# Autodesk Inventor assembly: A000
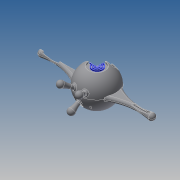
[picture p0: Inventor's stored thumbnail of the model, 180x180]
Saved by Autodesk Inventor 2017 (Build 210142000, 142)
## iProperties
Created: 2018-10-19
Part Number: A000
Document SubType Name: Assembly
Designer: Gilles Mottiez
Description: Prototype v2.0 Visible Energy
Author: Gilles Mottiez
## Documents named in this file (20)
- C:\Users\Gilles Mottiez\Documents\HES\I5_6\PGA\GitHubInventor\visibleEnergy_2.iam
- visibleEnergy_2.iam
- C:\Users\Gilles Mottiez\Documents\HES\I5_6\PGA\GitHubInventor\body_face_modif.ipt
- C:\Users\Gilles Mottiez\Documents\HES\I5_6\PGA\GitHubInventor\plateforme_rpi_servo.iam
- C:\Users\Gilles Mottiez\Documents\HES\I5_6\PGA\GitHubInventor\display_7seg.ipt
- C:\Users\Gilles Mottiez\Documents\HES\I5_6\PGA\GitHubInventor\arbre.ipt
- arbre.ipt
- C:\Users\Gilles Mottiez\Documents\HES\I5_6\PGA\GitHubInventor\palier_face.ipt
- palier_face.ipt
- C:\Users\Gilles Mottiez\Documents\HES\I5_6\PGA\GitHubInventor\body_dos.ipt
- C:\Users\Gilles Mottiez\Documents\HES\I5_6\PGA\GitHubInventor\axe.ipt
- axe.ipt
- C:\Users\Gilles Mottiez\Documents\HES\I5_6\PGA\GitHubInventor\ressort.ipt
- C:\Users\Gilles Mottiez\Documents\HES\I5_6\PGA\GitHubInventor\pieds.ipt
- C:\Users\Gilles Mottiez\Documents\HES\I5_6\PGA\GitHubInventor\bras_osc_dos.ipt
- bras_osc_dos.ipt
- C:\Users\Gilles Mottiez\Documents\HES\I5_6\PGA\GitHubInventor\bras_osc_front.ipt
- C:\Users\Gilles Mottiez\Documents\HES\I5_6\PGA\GitHubInventor\goupille_ressort.ipt
- goupille_ressort.ipt
- C:\Users\Gilles Mottiez\Documents\HES\I5_6\PGA\GitHubInventor\vis_blocage_arbre.ipt
## Components (17 placed, 13 different names)
1. body_face_modif:1 — Placage:1, Placage:2, Logement:1, Logement:2, Logement:4, Placage:3, Logement:9, Logement:11, Placage:6, Logement:22, Angle:3
2. plateforme_rpi_servo:1 [sub-assembly] — Placage:1, Placage:2, Logement:3, Logement:12, Logement:13, Logement:14, Logement:15, Logement:16, Logement:17, Logement:18, Logement:19, Angle:3
3. display_7seg:1 — Logement:1, Logement:2
4. arbre:1 — Logement:3, Logement:8, Placage:4, Placage:5, Logement:21
5. palier_face:1 — Logement:4
6. body_dos:1 — Logement:7, Logement:10, Placage:6, Logement:22, Angle:2
7. axe:1 — Logement:7
8. ressort:1 — Placage:3, Logement:8, Logement:20, Placage:4
9. pieds:1 — Logement:11
10. pieds:2 — Logement:9
11. pieds:3 — Logement:10, Angle:2
12. bras_osc_dos:1 — Logement:16, Logement:17
13. bras_osc_front:2 — Logement:14, Logement:15
14. bras_osc_dos:3 — Logement:18, Logement:19
15. bras_osc_front:4 — Logement:12, Logement:13
16. goupille_ressort:1 — Logement:20
17. vis_blocage_arbre:1 — Placage:5, Logement:21
## Relationships (28: Insert 20, Mate 6, Angle 2)
- Placage:1 [Mate]: body_face_modif:1 ↔ plateforme_rpi_servo:1
- Placage:2 [Mate]: body_face_modif:1 ↔ plateforme_rpi_servo:1
- Logement:1 [Insert]: body_face_modif:1 ↔ display_7seg:1
- Logement:2 [Insert]: body_face_modif:1 ↔ display_7seg:1
- Logement:3 [Insert]: plateforme_rpi_servo:1 ↔ arbre:1
- Logement:4 [Insert]: body_face_modif:1 ↔ palier_face:1
- Logement:7 [Insert]: body_dos:1 ↔ axe:1
- Placage:3 [Mate]: body_face_modif:1 ↔ ressort:1
- Logement:8 [Insert]: arbre:1 ↔ ressort:1
- Logement:9 [Insert]: body_face_modif:1 ↔ pieds:2
- Logement:10 [Insert]: body_dos:1 ↔ pieds:3
- Logement:11 [Insert]: body_face_modif:1 ↔ pieds:1
- Logement:12 [Insert]: plateforme_rpi_servo:1 ↔ bras_osc_front:4
- Logement:13 [Insert]: plateforme_rpi_servo:1 ↔ bras_osc_front:4
- Logement:14 [Insert]: plateforme_rpi_servo:1 ↔ bras_osc_front:2
- Logement:15 [Insert]: plateforme_rpi_servo:1 ↔ bras_osc_front:2
- Logement:16 [Insert]: plateforme_rpi_servo:1 ↔ bras_osc_dos:1
- Logement:17 [Insert]: plateforme_rpi_servo:1 ↔ bras_osc_dos:1
- Logement:18 [Insert]: plateforme_rpi_servo:1 ↔ bras_osc_dos:3
- Logement:19 [Insert]: plateforme_rpi_servo:1 ↔ bras_osc_dos:3
- Logement:20 [Insert]: ressort:1 ↔ goupille_ressort:1
- Placage:4 [Mate]: arbre:1 ↔ ressort:1
- Placage:5 [Mate]: arbre:1 ↔ vis_blocage_arbre:1
- Logement:21 [Insert] (1 mm): arbre:1 ↔ vis_blocage_arbre:1
- Placage:6 [Mate]: body_face_modif:1 ↔ body_dos:1
- Logement:22 [Insert]: body_face_modif:1 ↔ body_dos:1
- Angle:2 (0 deg): body_dos:1 ↔ pieds:3
- Angle:3 (0 deg): body_face_modif:1 ↔ plateforme_rpi_servo:1
